# Autodesk Inventor assembly: Horn with Flange
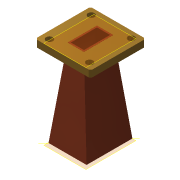
[picture p0: Inventor's stored thumbnail of the model, 180x180]
Saved by Autodesk Inventor 2015 SP1 (Build 190203100, 203)
## iProperties
Created: 2016-04-07
Part Number: Horn with Flange
Document SubType Name: Assembly
Designer: jad211
Author: jad211
## Documents named in this file (3)
- C:\ColdMatter\CADFiles\EDM Machine\Detection Region\Microwave Horn Assembly\Horn with Flange.iam
- C:\ColdMatter\CADFiles\EDM Machine\Pumping Region\Pumping Region\NewHorn.ipt
- C:\ColdMatter\CADFiles\EDM Machine\Pumping Region\Pumping Region\WG18FLANGE.ipt
## Components (2 placed, 2 different names)
1. NewHorn:1 — Mate:1, Mate:2
2. WG18FLANGE:1 — Mate:1, Mate:2
## Relationships (2: Mate 2)
- Mate:1: NewHorn:1 ↔ WG18FLANGE:1
- Mate:2: NewHorn:1 ↔ WG18FLANGE:1
